# Autodesk Inventor assembly: Slider
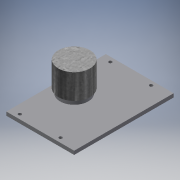
[picture p0: Inventor's stored thumbnail of the model, 180x180]
Saved by Autodesk Inventor 2019 (Build 230136000, 136)
## iProperties
Created: 2020-04-04
Part Number: Slider
Document SubType Name: Assembly
Designer: james
Author: james
## Documents named in this file (3)
- F:\JimsRobot\FIRSTRobots\Design\TornadoPlatypus\Slider.iam
- F:\JimsRobot\FIRSTRobots\Design\TornadoPlatypus\Slider.ipt
- F:\JimsRobot\FIRSTRobots\Design\TornadoPlatypus\HudsonRoller.ipt
## Components (2 placed, 2 different names)
1. Slider:1 — Mate:1, Mate:2
2. HudsonRoller:1 — Mate:1, Mate:2
## Relationships (2: Mate 2)
- Mate:1: Slider:1 ↔ HudsonRoller:1
- Mate:2: Slider:1 ↔ HudsonRoller:1
